# Autodesk Inventor assembly: Leg_joint_roll_yaw
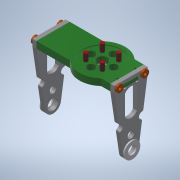
[picture p0: Inventor's stored thumbnail of the model, 180x180]
Saved by Autodesk Inventor 2020 (Build 240168000, 168)
## iProperties
Created: 2016-05-01
Part Number: Leg_joint_roll_yaw
Document SubType Name: Assembly
Designer: hiroaki
Mass: 101.489 g
Surface Area: 218.083 cm^2
Volume: 17.9148 cm^3
Density: 5.6651 g/cm^3
Author: hiroaki
## Documents named in this file (6)
- C:\Users\Masato\Desktop\OpenPlatform_ver3_0 - Ver4_1branch\LowerBody\Leg_joit\Leg_joint_roll_yaw.iam
- C:\Users\Masato\Desktop\OpenPlatform_ver3_0 - Ver4_1branch\LowerBody\Leg_joit\Leg_joint_yaw_frame.ipt
- C:\Users\Masato\Desktop\OpenPlatform_ver3_0 - Ver4_1branch\Ready_Made\Screw\M3-10.ipt
- C:\Users\Masato\Desktop\OpenPlatform_ver3_0 - Ver4_1branch\Ready_Made\Screw\M3-6.ipt
- C:\Users\Masato\Desktop\OpenPlatform_ver3_0 - Ver4_1branch\LowerBody\Leg_joit\Leg_joint_slider_frame.ipt
- C:\Users\Masato\Desktop\OpenPlatform_ver3_0 - Ver4_1branch\Ready_Made\TT-0612-10.ipt
## Components (13 placed, 5 different names)
1. Leg_joint_yaw_frame:1 — 挿入:1, 挿入:2, 挿入:3, 挿入:4, 挿入:5, 挿入:6, 挿入:7, 挿入:8, フラッシュ:1, フラッシュ:2, メイト:1
2. Leg_joint_slider_frame:1 — 挿入:1, 挿入:2, 挿入:9, 挿入:10, 挿入:13
3. Leg_joint_slider_frame:2 — 挿入:3, 挿入:4, 挿入:11, 挿入:12, 挿入:14
4. M3-10:1 — 挿入:5
5. M3-10:2 — 挿入:6
6. M3-10:3 — 挿入:7
7. M3-10:4 — 挿入:8
8. M3-6:1 — 挿入:10
9. M3-6:2 — 挿入:9
10. M3-6:3 — 挿入:12
11. M3-6:4 — 挿入:11
12. TT-0612-10:1 — 挿入:13
13. TT-0612-10:2 — 挿入:14
## Relationships (17: Insert 14, Flush 2, Mate 1)
- 挿入:1 [Insert]: Leg_joint_yaw_frame:1 ↔ Leg_joint_slider_frame:1
- 挿入:2 [Insert]: Leg_joint_yaw_frame:1 ↔ Leg_joint_slider_frame:1
- 挿入:3 [Insert]: Leg_joint_yaw_frame:1 ↔ Leg_joint_slider_frame:2
- 挿入:4 [Insert]: Leg_joint_yaw_frame:1 ↔ Leg_joint_slider_frame:2
- 挿入:5 [Insert]: Leg_joint_yaw_frame:1 ↔ M3-10:1
- 挿入:6 [Insert]: Leg_joint_yaw_frame:1 ↔ M3-10:2
- 挿入:7 [Insert]: Leg_joint_yaw_frame:1 ↔ M3-10:3
- 挿入:8 [Insert]: Leg_joint_yaw_frame:1 ↔ M3-10:4
- 挿入:9 [Insert]: Leg_joint_slider_frame:1 ↔ M3-6:2
- 挿入:10 [Insert]: Leg_joint_slider_frame:1 ↔ M3-6:1
- 挿入:11 [Insert]: Leg_joint_slider_frame:2 ↔ M3-6:4
- 挿入:12 [Insert]: Leg_joint_slider_frame:2 ↔ M3-6:3
- 挿入:13 [Insert]: Leg_joint_slider_frame:1 ↔ TT-0612-10:1
- 挿入:14 [Insert]: Leg_joint_slider_frame:2 ↔ TT-0612-10:2
- フラッシュ:1 [Flush]: Leg_joint_yaw_frame:1
- フラッシュ:2 [Flush]: Leg_joint_yaw_frame:1
- メイト:1 [Mate]: Leg_joint_yaw_frame:1
